# Autodesk Inventor assembly: rowing_steering
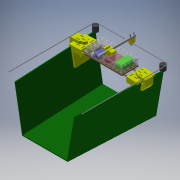
[picture p0: Inventor's stored thumbnail of the model, 180x180]
Saved by Autodesk Inventor 2019 (Build 230136000, 136)
## iProperties
Created: 2019-01-31
Part Number: rowing_steering
Document SubType Name: Assembly
Designer: suchanek
Author: suchanek
## Documents named in this file (18)
- D:\suchanek\programming\rowing_steering\rowing_steering.iam
- D:\suchanek\programming\rowing_steering\boat_segment.ipt
- D:\suchanek\programming\rowing_steering\holder_inner.ipt
- D:\suchanek\programming\rowing_steering\holder_bar.ipt
- D:\suchanek\programming\rowing_steering\case_base.ipt
- D:\suchanek\programming\rowing_steering\holder_outer.ipt
- D:\suchanek\programming\rowing_steering\servo.ipt
- D:\suchanek\programming\rowing_steering\case_back.ipt
- D:\suchanek\programming\rowing_steering\case_top.ipt
- D:\suchanek\programming\rowing_steering\case_front.ipt
- D:\suchanek\programming\rowing_steering\case_side.ipt
- D:\suchanek\programming\rowing_steering\arduino-uno.snapshot.3\arduino uno.iam
- D:\suchanek\programming\rowing_steering\battery.ipt
- D:\suchanek\programming\rowing_steering\arm.ipt
- D:\suchanek\programming\rowing_steering\gripper.ipt
- D:\suchanek\programming\rowing_steering\gripper_bolt.ipt
- D:\suchanek\programming\rowing_steering\arm_safe.ipt
- D:\suchanek\programming\rowing_steering\servo_piece.ipt
## Components (21 placed, 17 different names)
1. boat_segment:1 — Mate:1, Mate:2, Angle:1, Mate:35
2. holder_inner:1 — Mate:1, Symmetry:1, Symmetry:2, Mate:2, Symmetry:3, Mate:3, Tangent:1, Mate:4, Tangent:2
3. holder_inner:2 — Symmetry:1, Symmetry:2, Symmetry:3, Mate:6, Angle:4, Tangent:5
4. holder_bar:1 — Angle:2, Mate:4, Tangent:2, Mate:13, Angle:5, Tangent:6, Tangent:8
5. holder_bar:2 — Angle:1, Mate:3, Tangent:1, Angle:2, Tangent:7
6. case_base:1 — Mate:13, Angle:5, Tangent:6, Tangent:7, Tangent:8, Mate:14, Mate:15, Mate:17, Angle:6, Flush:1, Mate:19, Mate:21, Mate:22, Mate:23, Mate:24, Mate:25, Angle:7, Mate:27, Tangent:9
7. holder_outer:1 — Symmetry:4, Symmetry:5, Symmetry:6
8. holder_outer:2 — Mate:6, Angle:4, Tangent:5, Symmetry:4, Symmetry:5, Symmetry:6
9. servo:1 — Mate:16, Mate:17, Angle:6, Rotational:1
10. case_back:1 — Mate:11, Mate:12, Mate:14, Mate:15, Mate:18
11. case_top:1 — Mate:11, Mate:12, Mate:16, Flush:1, Mate:18, Flush:2, Mate:20, Flush:3, Flush:4, Flush:5, Angle:8
12. case_front:1 — Flush:2, Mate:19, Mate:20, Mate:26
13. case_side:1 — Mate:21, Mate:22, Flush:3
14. case_side:2 — Flush:4, Mate:23, Flush:5
15. arduino uno:1 [sub-assembly] — Mate:24, Mate:25, Angle:7
16. battery:1 — Mate:26, Mate:27, Tangent:9
17. arm:1 — Angle:8, Mate:31, Flush:7, Mate:32, Mate:37, Mate:38
18. gripper:1 — Mate:31, Flush:7, Mate:32, Mate:33, Mate:34, Mate:35, Mate:36
19. gripper_bolt:1 — Mate:33, Mate:34, Mate:36
20. arm_safe:1 — Mate:39, Mate:40, Mate:41
21. servo_piece:1 — Rotational:1, Mate:37, Mate:38, Mate:39, Mate:40, Mate:41
## Relationships (60: Mate 33, Angle 7, Tangent 7, Symmetry 6, Flush 6, RevoluteJoint 1)
- Mate:1: boat_segment:1 ↔ holder_inner:1
- Symmetry:1: holder_inner:1 ↔ holder_inner:2
- Symmetry:2: holder_inner:1 ↔ holder_inner:2
- Mate:2: boat_segment:1 ↔ holder_inner:1
- Symmetry:3: holder_inner:1 ↔ holder_inner:2
- Angle:1 (0 deg): boat_segment:1 ↔ holder_bar:2
- Mate:3: holder_inner:1 ↔ holder_bar:2
- Tangent:1: holder_inner:1 ↔ holder_bar:2
- Angle:2 (0 deg): holder_bar:1 ↔ holder_bar:2
- Mate:4: holder_inner:1 ↔ holder_bar:1
- Tangent:2: holder_inner:1 ↔ holder_bar:1
- Mate:6: holder_inner:2 ↔ holder_outer:2
- Angle:4 (0 deg): holder_inner:2 ↔ holder_outer:2
- Tangent:5: holder_inner:2 ↔ holder_outer:2
- Symmetry:4: holder_outer:1 ↔ holder_outer:2
- Symmetry:5: holder_outer:1 ↔ holder_outer:2
- Symmetry:6: holder_outer:1 ↔ holder_outer:2
- Mate:11: case_back:1 ↔ case_top:1
- Mate:12: case_back:1 ↔ case_top:1
- Mate:13: holder_bar:1 ↔ case_base:1
- Angle:5 (0 deg): holder_bar:1 ↔ case_base:1
- Tangent:6: holder_bar:1 ↔ case_base:1
- Tangent:7: holder_bar:2 ↔ case_base:1
- Tangent:8: holder_bar:1 ↔ case_base:1
- Mate:14: case_base:1 ↔ case_back:1
- Mate:15: case_base:1 ↔ case_back:1
- Mate:16: servo:1 ↔ case_top:1
- Mate:17: case_base:1 ↔ servo:1
- Angle:6 (0 deg): case_base:1 ↔ servo:1
- Flush:1: case_base:1 ↔ case_top:1
- Mate:18: case_back:1 ↔ case_top:1
- Flush:2: case_top:1 ↔ case_front:1
- Mate:19: case_base:1 ↔ case_front:1
- Mate:20: case_top:1 ↔ case_front:1
- Mate:21: case_base:1 ↔ case_side:1
- Mate:22: case_base:1 ↔ case_side:1
- Flush:3: case_top:1 ↔ case_side:1
- Flush:4: case_top:1 ↔ case_side:2
- Mate:23: case_base:1 ↔ case_side:2
- Flush:5: case_top:1 ↔ case_side:2
- Mate:24 (2 mm): case_base:1 ↔ arduino uno:1
- Mate:25: case_base:1 ↔ arduino uno:1
- Angle:7 (0 deg): case_base:1 ↔ arduino uno:1
- Mate:26: case_front:1 ↔ battery:1
- Mate:27: case_base:1 ↔ battery:1
- Tangent:9: case_base:1 ↔ battery:1
- Angle:8 (0 deg): case_top:1 ↔ arm:1
- Mate:31: arm:1 ↔ gripper:1
- Flush:7: arm:1 ↔ gripper:1
- Mate:32: arm:1 ↔ gripper:1
- Mate:33: gripper:1 ↔ gripper_bolt:1
- Mate:34: gripper:1 ↔ gripper_bolt:1
- Mate:35 (-15 mm): boat_segment:1 ↔ gripper:1
- Mate:36: gripper:1 ↔ gripper_bolt:1
- Rotational:1 [RevoluteJoint]: servo:1 ↔ servo_piece:1
- Mate:37: arm:1 ↔ servo_piece:1
- Mate:38: arm:1 ↔ servo_piece:1
- Mate:39: arm_safe:1 ↔ servo_piece:1
- Mate:40: arm_safe:1 ↔ servo_piece:1
- Mate:41: arm_safe:1 ↔ servo_piece:1
